# Autodesk Inventor assembly: toaster
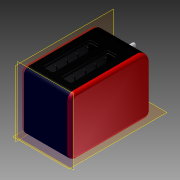
[picture p0: Inventor's stored thumbnail of the model, 180x180]
Saved by Autodesk Inventor 2015 (Build 190159000, 159)
## iProperties
Created: 2015-10-18
Part Number: toaster
Document SubType Name: Assembly
Designer: omae
Author: omae
## Documents named in this file (2)
- C:\Users\omae\Desktop\研究室\論文・資料\ROS\kitchen\stl\toaster.iam
- C:\Users\omae\Desktop\研究室\論文・資料\ROS\kitchen\zip\pantone-toast-maker-1.snapshot.2\pantoaster\panToaster_glass.iam
## Components (1 placed, 1 different names)
1. panToaster_glass:1 [sub-assembly] — メイト:1, メイト:2, メイト:3
## Relationships (3: Mate 3)
- メイト:1 [Mate]: panToaster_glass:1
- メイト:2 [Mate]: panToaster_glass:1
- メイト:3 [Mate]: panToaster_glass:1
